# Autodesk Inventor assembly: Hoja Oculta
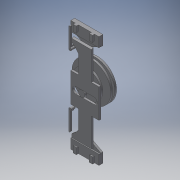
[picture p0: Inventor's stored thumbnail of the model, 180x180]
Saved by Autodesk Inventor 2017 (Build 210142000, 142)
## iProperties
Created: 2017-01-19
Part Number: Hoja Oculta
Document SubType Name: Assembly
Designer: A. Matías Quezada
Author: A. Matías Quezada
## Documents named in this file (12)
- D:\repos\3D\Hoja Oculta\Prototipo\Hoja Oculta.iam
- D:\repos\3D\Hoja Oculta\Prototipo\Base.ipt
- D:\repos\3D\Hoja Oculta\Prototipo\Hoja.ipt
- D:\repos\3D\Hoja Oculta\Prototipo\Tirador.ipt
- D:\repos\3D\Hoja Oculta\Prototipo\Deslizador.ipt
- D:\repos\3D\Hoja Oculta\Prototipo\Parametros.ipt
- D:\repos\3D\Hoja Oculta\Prototipo\Traba.ipt
- D:\repos\3D\Hoja Oculta\Prototipo\Traba_MIR.ipt
- D:\repos\3D\Hoja Oculta\Prototipo\Rueda Interna.ipt
- D:\repos\3D\Hoja Oculta\Prototipo\Tapa.ipt
- D:\repos\3D\Hoja Oculta\Prototipo\Rueda Externa.ipt
- D:\repos\3D\Hoja Oculta\Prototipo\Rueda Superior.ipt
## Components (11 placed, 10 different names)
1. Base:1 — Movimiento Hoja, Slider:4, Slider:5, Slider:6, Rotational:1, Rotational:2, Mate:10, Rigid:1
2. Hoja:1 — Movimiento Hoja, Hoja-Tirador2, Hoja-Tirador1
3. Tirador:1 — Slider:6, Deslizador-Tirador1, Hoja-Tirador1
4. Tirador:2 — Slider:5, Deslizador-Tirador2, Hoja-Tirador2
5. Deslizador:1 — Slider:4, Deslizador-Tirador2, Deslizador-Tirador1, Tangent:1, Mate:9
6. Traba:1 — Rotational:1
7. Traba_MIR:1 — Rotational:2
8. Rueda Interna:1 — Tangent:1, Mate:9, Mate:10, Rigid:2
9. Tapa:1 — Rigid:1, Cylindrical:1
10. Rueda Externa:1 — Rigid:2, Cylindrical:1, Rigid:3
11. Rueda Superior:1 — Rigid:3
## Relationships (17: Mate 6, TranslationJoint 4, WeldJoint 3, RevoluteJoint 2, Tangent 1, CylindricalJoint 1)
- Movimiento Hoja [TranslationJoint] (1 mm): Base:1 ↔ Hoja:1
- Slider:4 [TranslationJoint]: Base:1 ↔ Deslizador:1
- Slider:5 [TranslationJoint]: Base:1 ↔ Tirador:2
- Deslizador-Tirador2 [Mate]: Tirador:2 ↔ Deslizador:1
- Slider:6 [TranslationJoint]: Base:1 ↔ Tirador:1
- Deslizador-Tirador1 [Mate]: Tirador:1 ↔ Deslizador:1
- Hoja-Tirador2 [Mate]: Hoja:1 ↔ Tirador:2
- Hoja-Tirador1 [Mate]: Hoja:1 ↔ Tirador:1
- Rotational:1 [RevoluteJoint]: Base:1 ↔ Traba:1
- Rotational:2 [RevoluteJoint]: Base:1 ↔ Traba_MIR:1
- Tangent:1: Deslizador:1 ↔ Rueda Interna:1
- Mate:9: Deslizador:1 ↔ Rueda Interna:1
- Mate:10 (22 mm): Base:1 ↔ Rueda Interna:1
- Rigid:1 [WeldJoint]: Base:1 ↔ Tapa:1
- Rigid:2 [WeldJoint]: Rueda Interna:1 ↔ Rueda Externa:1
- Cylindrical:1: Tapa:1 ↔ Rueda Externa:1
- Rigid:3 [WeldJoint]: Rueda Externa:1 ↔ Rueda Superior:1
## Named parameters: movimiento_deslizador = 28.6 mm, movimiento_hoja = 177.4 mm
